# Autodesk Inventor assembly: Hand Assem
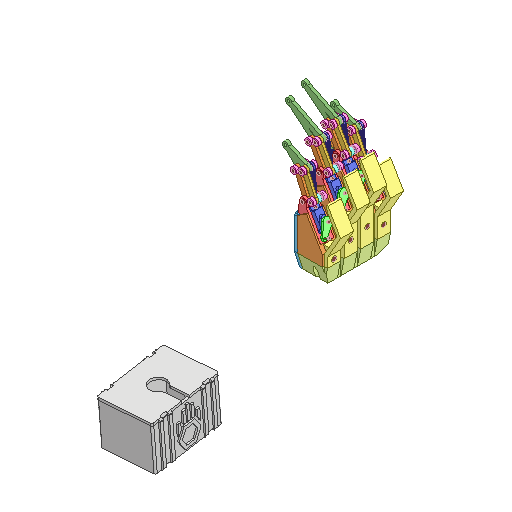
[picture p0: Inventor's stored thumbnail of the model, 512x512]
Saved by Autodesk Inventor 2025.1 (Build 291241020, 241B)
## iProperties
Created: 2024-11-29
Part Number: Hand Assem
Document SubType Name: Assembly
Designer: alexa
Author: alexa
## Documents named in this file (23)
- D:\CAD\Inventor\Bio Kettering Hand\Liv Mas 1.0\Hand Assem.iam
- D:\CAD\Inventor\Bio Kettering Hand\Liv Mas 1.0\PALM 1.ipt
- D:\CAD\Inventor\Bio Kettering Hand\Liv Mas 1.0\KNUCKLE 1.ipt
- D:\CAD\Inventor\Bio Kettering Hand\Liv Mas 1.0\PALM 2.ipt
- D:\CAD\Inventor\Bio Kettering Hand\Liv Mas 1.0\PALM 3.ipt
- D:\CAD\Inventor\Bio Kettering Hand\Liv Mas 1.0\PALM 4.ipt
- D:\CAD\Inventor\Bio Kettering Hand\Liv Mas 1.0\KNUCKLE 2.ipt
- D:\CAD\Inventor\Bio Kettering Hand\Liv Mas 1.0\KNUCKLE 3.ipt
- D:\CAD\Inventor\Bio Kettering Hand\Liv Mas 1.0\KNUCKLE 4.ipt
- D:\CAD\Inventor\Bio Kettering Hand\Liv Mas 1.0\Finger Assem.iam
- D:\CAD\Inventor\Bio Kettering Hand\Liv Mas 1.0\Servo.ipt
- D:\CAD\Inventor\Bio Kettering Hand\Liv Mas 1.0\Thumb Assem.iam
- D:\CAD\Inventor\Bio Kettering Hand\Liv Mas 1.0\Thumb Base2.ipt
- D:\CAD\Inventor\Bio Kettering Hand\Liv Mas 1.0\Wrist Base.ipt
- D:\CAD\Inventor\Bio Kettering Hand\Liv Mas 1.0\Palm.ipt
- D:\CAD\Inventor\Bio Kettering Hand\Liv Mas 1.0\Screw BIG 3.ipt
- D:\CAD\Inventor\Bio Kettering Hand\Liv Mas 1.0\Screw PROP.ipt
- D:\CAD\Inventor\Bio Kettering Hand\Liv Mas 1.0\Finger Assem 2.iam
- D:\CAD\Inventor\Bio Kettering Hand\Liv Mas 1.0\Finger Assem 3.iam
- D:\CAD\Inventor\Bio Kettering Hand\Liv Mas 1.0\Finger Assem 4.iam
- D:\CAD\Inventor\Bio Kettering Hand\Liv Mas 1.0\Hand Stand.ipt
- D:\CAD\Inventor\Bio Kettering Hand\Liv Mas 1.0\Janus wire holder.ipt
- D:\CAD\Inventor\Bio Kettering Hand\Liv Mas 1.0\Janus wire holder lid.ipt
## Components (44 placed, 22 different names)
1. KNUCKLE 1:1 — Flush:7, Mate:4, Mate:8, Rigid:3
2. KNUCKLE 2:1 — Flush:10, Mate:5, Mate:9, Rotational:16
3. KNUCKLE 3:1 — Flush:9, Mate:6, Mate:10, Rotational:15
4. KNUCKLE 4:1 — Flush:8, Mate:7, Mate:11, Rotational:14
5. PALM 1:1 — Mate:1, Flush:1, Flush:2, Flush:7, Mate:4, Mate:8, Mate:12, Mate:13, Mate:14, Flush:14, Mate:30
6. PALM 2:1 — Mate:1, Flush:1, Flush:2, Mate:2, Flush:3, Flush:4, Flush:8, Flush:9, Mate:5, Mate:9, Mate:34, Mate:35, Mate:36
7. PALM 3:1 — Mate:2, Flush:3, Flush:4, Flush:5, Flush:6, Mate:3, Flush:10, Mate:6, Mate:10, Mate:37, Mate:38, Mate:39
8. PALM 4:1 — Flush:5, Flush:6, Mate:3, Mate:7, Mate:11, Mate:24, Mate:25, Flush:11, Flush:12, Mate:31, Mate:32, Mate:33
9. Finger Assem:1 [sub-assembly] — Mate:12, Mate:13, Mate:14, Rotational:20
10. Servo:2 — Rotational:1, Mate:26, Mate:27, Mate:28
11. Thumb Assem:1 [sub-assembly] — Rotational:1
12. Thumb Base2:1 — Mate:24, Mate:25, Flush:11, Mate:26, Mate:27, Mate:28, Flush:15, Rotational:9, Rotational:13
13. Wrist Base:1 — Flush:12, Rotational:2, Rotational:3, Rotational:4, Rigid:1, Rotational:5, Rotational:6, Rotational:7, Rotational:21
14. Palm:1 — Flush:14, Mate:30, Flush:15, Rotational:8, Rigid:2, Rotational:10, Rotational:11, Rotational:12, Rotational:22, Angle:1
15. Screw BIG 3:1 — Rotational:2
16. Screw BIG 3:2 — Rotational:4
17. Screw BIG 3:3 — Rotational:3
18. Screw BIG 3:4 — Rotational:5
19. Screw BIG 3:5 — Rotational:7
20. Screw BIG 3:6 — Rotational:6
21. Screw BIG 3:7 — Rigid:1
22. Screw BIG 3:8 — Rotational:8
23. Screw BIG 3:9 — Rotational:12
24. Screw BIG 3:10 — Rigid:2
25. Screw BIG 3:11 — Rotational:10
26. Screw BIG 3:12 — Rotational:11
27. Screw BIG 3:13 — Rotational:9
28. Screw BIG 3:14 — Rotational:13
29. Screw BIG 3:15 — Rotational:14
30. Screw BIG 3:16 — Rotational:15
31. Screw BIG 3:17 — Rigid:3
32. Screw BIG 3:18 — Rotational:16
33. Screw PROP:1
34. Screw PROP:2
35. Screw PROP:3 — Rotational:20
36. Screw PROP:4
37. Screw BIG 3:19 — Rotational:21
38. Finger Assem 2:1 [sub-assembly] — Mate:34, Mate:35, Mate:36
39. Finger Assem 3:1 [sub-assembly] — Mate:37, Mate:38, Mate:39
40. Finger Assem 4:1 [sub-assembly] — Mate:31, Mate:32, Mate:33
41. Screw BIG 3:20 — Rotational:22
42. Hand Stand:1 — Angle:1
43. Janus wire holder:1 — Mate:40, Flush:16, Flush:17
44. Janus wire holder lid:1 — Mate:40, Flush:16, Flush:17
## Relationships (69: Mate 30, RevoluteJoint 19, Flush 16, WeldJoint 3, Angle 1)
- Mate:1: PALM 1:1 ↔ PALM 2:1
- Flush:1: PALM 1:1 ↔ PALM 2:1
- Flush:2: PALM 1:1 ↔ PALM 2:1
- Mate:2: PALM 2:1 ↔ PALM 3:1
- Flush:3: PALM 2:1 ↔ PALM 3:1
- Flush:4: PALM 2:1 ↔ PALM 3:1
- Flush:5: PALM 3:1 ↔ PALM 4:1
- Flush:6: PALM 3:1 ↔ PALM 4:1
- Mate:3: PALM 3:1 ↔ PALM 4:1
- Flush:7: KNUCKLE 1:1 ↔ PALM 1:1
- Flush:8: KNUCKLE 4:1 ↔ PALM 2:1
- Flush:9: KNUCKLE 3:1 ↔ PALM 2:1
- Flush:10: KNUCKLE 2:1 ↔ PALM 3:1
- Mate:4: KNUCKLE 1:1 ↔ PALM 1:1
- Mate:5: KNUCKLE 2:1 ↔ PALM 2:1
- Mate:6: KNUCKLE 3:1 ↔ PALM 3:1
- Mate:7: KNUCKLE 4:1 ↔ PALM 4:1
- Mate:8: KNUCKLE 1:1 ↔ PALM 1:1
- Mate:9: KNUCKLE 2:1 ↔ PALM 2:1
- Mate:10: KNUCKLE 3:1 ↔ PALM 3:1
- Mate:11: KNUCKLE 4:1 ↔ PALM 4:1
- Mate:12: PALM 1:1 ↔ Finger Assem:1
- Mate:13: PALM 1:1 ↔ Finger Assem:1
- Mate:14: PALM 1:1 ↔ Finger Assem:1
- Rotational:1 [RevoluteJoint]: Servo:2 ↔ Thumb Assem:1
- Mate:24: PALM 4:1 ↔ Thumb Base2:1
- Mate:25: PALM 4:1 ↔ Thumb Base2:1
- Flush:11: PALM 4:1 ↔ Thumb Base2:1
- Mate:26: Servo:2 ↔ Thumb Base2:1
- Mate:27: Servo:2 ↔ Thumb Base2:1
- Mate:28: Servo:2 ↔ Thumb Base2:1
- Flush:12: PALM 4:1 ↔ Wrist Base:1
- Flush:14: PALM 1:1 ↔ Palm:1
- Mate:30: PALM 1:1 ↔ Palm:1
- Flush:15: Thumb Base2:1 ↔ Palm:1
- Rotational:2 [RevoluteJoint]: Wrist Base:1 ↔ Screw BIG 3:1
- Rotational:3 [RevoluteJoint]: Wrist Base:1 ↔ Screw BIG 3:3
- Rotational:4 [RevoluteJoint]: Wrist Base:1 ↔ Screw BIG 3:2
- Rigid:1 [WeldJoint]: Wrist Base:1 ↔ Screw BIG 3:7
- Rotational:5 [RevoluteJoint]: Wrist Base:1 ↔ Screw BIG 3:4
- Rotational:6 [RevoluteJoint]: Wrist Base:1 ↔ Screw BIG 3:6
- Rotational:7 [RevoluteJoint]: Wrist Base:1 ↔ Screw BIG 3:5
- Rotational:8 [RevoluteJoint]: Palm:1 ↔ Screw BIG 3:8
- Rotational:9 [RevoluteJoint]: Thumb Base2:1 ↔ Screw BIG 3:13
- Rigid:2 [WeldJoint]: Palm:1 ↔ Screw BIG 3:10
- Rotational:10 [RevoluteJoint]: Palm:1 ↔ Screw BIG 3:11
- Rotational:11 [RevoluteJoint]: Palm:1 ↔ Screw BIG 3:12
- Rotational:12 [RevoluteJoint]: Palm:1 ↔ Screw BIG 3:9
- Rotational:13 [RevoluteJoint]: Thumb Base2:1 ↔ Screw BIG 3:14
- Rotational:14 [RevoluteJoint]: KNUCKLE 4:1 ↔ Screw BIG 3:15
- Rotational:15 [RevoluteJoint]: KNUCKLE 3:1 ↔ Screw BIG 3:16
- Rotational:16 [RevoluteJoint]: KNUCKLE 2:1 ↔ Screw BIG 3:18
- Rigid:3 [WeldJoint]: KNUCKLE 1:1 ↔ Screw BIG 3:17
- Rotational:20 [RevoluteJoint]: Finger Assem:1 ↔ Screw PROP:3
- Rotational:21 [RevoluteJoint]: Wrist Base:1 ↔ Screw BIG 3:19
- Mate:31: PALM 4:1 ↔ Finger Assem 4:1
- Mate:32: PALM 4:1 ↔ Finger Assem 4:1
- Mate:33: PALM 4:1 ↔ Finger Assem 4:1
- Mate:34: PALM 2:1 ↔ Finger Assem 2:1
- Mate:35: PALM 2:1 ↔ Finger Assem 2:1
- Mate:36: PALM 2:1 ↔ Finger Assem 2:1
- Mate:37: PALM 3:1 ↔ Finger Assem 3:1
- Mate:38: PALM 3:1 ↔ Finger Assem 3:1
- Mate:39: PALM 3:1 ↔ Finger Assem 3:1
- Rotational:22 [RevoluteJoint]: Palm:1 ↔ Screw BIG 3:20
- Angle:1 (0 deg): Palm:1 ↔ Hand Stand:1
- Mate:40: Janus wire holder:1 ↔ Janus wire holder lid:1
- Flush:16: Janus wire holder:1 ↔ Janus wire holder lid:1
- Flush:17: Janus wire holder:1 ↔ Janus wire holder lid:1
